# Autodesk Inventor assembly: Dose
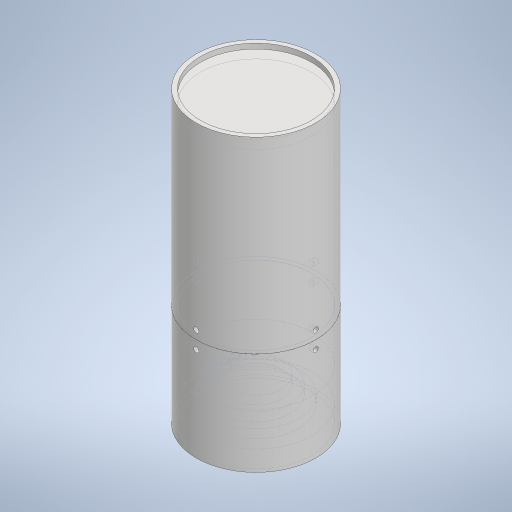
[picture p0: Inventor's stored thumbnail of the model, 512x512]
Saved by Autodesk Inventor 2024 (Build 280153000, 153)
## iProperties
Created: 2024-02-13
Part Number: Dose
Document SubType Name: Assembly
Designer: Daniel Nussbaum
Author: Daniel Nussbaum
## Documents named in this file (3)
- C:\GitHubDesktop\3d-model\dose\Dose.iam
- C:\GitHubDesktop\3d-model\dose\Grundkörper.ipt
- C:\GitHubDesktop\3d-model\dose\GrundkörperOben.ipt
## Components (2 placed, 2 different names)
1. Grundkörper:1 — Flush:1
2. GrundkörperOben:1 — Flush:1
## Relationships (1: Flush 1)
- Flush:1: Grundkörper:1 ↔ GrundkörperOben:1
